# Autodesk Inventor assembly: 42146-20-03
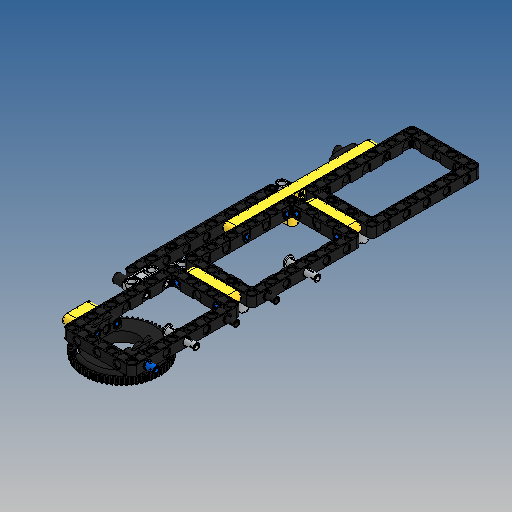
[picture p0: Inventor's stored thumbnail of the model, 512x512]
Saved by Autodesk Inventor 2025 (Build 290162010, 162A)
## iProperties
Created: 2024-11-22
Part Number: 42146-20-03
Material: Generisch
Document SubType Name: Assembly
Designer: hp.muther
Author: hp.muther
## Documents named in this file (14)
- D:\Inventor\Projekte\Muther\LEGO Technic\LEGO Technik - Raupenkran LR 13000 (42146)\42146-20-03.iam
- D:\Inventor\Projekte\Muther\LEGO Technic\LEGO Pieces\Rahmen, T-Stücke\39794-Black.ipt
- D:\Inventor\Projekte\Muther\LEGO Technic\LEGO Pieces\Pin's\2780-Black.ipt
- D:\Inventor\Projekte\Muther\LEGO Technic\LEGO Pieces\Pin's\6558-Blue.ipt
- D:\Inventor\Projekte\Muther\LEGO Technic\LEGO Pieces\Pin's\32054-LtBluishGray.ipt
- D:\Inventor\Projekte\Muther\LEGO Technic\LEGO Pieces\Lochbalken\32523-Yellow.ipt
- D:\Inventor\Projekte\Muther\LEGO Technic\LEGO Pieces\Lochbalken\32316-Yellow.ipt
- D:\Inventor\Projekte\Muther\LEGO Technic\LEGO Pieces\Lochbalken\32278-Yellow.ipt
- D:\Inventor\Projekte\Muther\LEGO Technic\LEGO Pieces\Lochbalken\771710-Black.ipt
- D:\Inventor\Projekte\Muther\LEGO Technic\LEGO Pieces\Lochbalken\40490-LtBluishGray.ipt
- D:\Inventor\Projekte\Muther\LEGO Technic\LEGO Pieces\Rund\18654-Black.ipt
- D:\Inventor\Projekte\Muther\LEGO Technic\LEGO Pieces\Verbindungselemente\48989-LtBluishGray.ipt
- D:\Inventor\Projekte\Muther\LEGO Technic\LEGO Pieces\Verbindungselemente\15461-Black.ipt
- D:\Inventor\Projekte\Muther\LEGO Technic\LEGO Pieces\Zahnrad\18938-BLACK.ipt
## Components (36 placed, 13 different names)
1. 39794-Black:1 — Einfügen:1, Einfügen:2, Einfügen:3, Einfügen:4, Passend:1, Einfügen:8, Einfügen:9, Passend:2, Passend:3, Einfügen:17, Passend:7
2. 2780-Black:1 — Einfügen:1
3. 6558-Blue:1 — Einfügen:2
4. 32054-LtBluishGray:1 — Einfügen:3
5. 18938-BLACK:1 — Einfügen:4, Passend:1
6. 32523-Yellow:1 — Einfügen:5, Einfügen:6, Einfügen:8
7. 6558-Blue:2 — Einfügen:6, Passend:3
8. 6558-Blue:3 — Einfügen:5
9. 6558-Blue:4 — Einfügen:11, Passend:4, Passend:7
10. 6558-Blue:5 — Einfügen:10
11. 39794-Black:2 — Einfügen:12, Passend:4, Einfügen:16, Passend:6, Einfügen:22, Einfügen:24, Einfügen:25, Einfügen:26, Einfügen:29, Einfügen:34
12. 32316-Yellow:1 — Einfügen:10, Einfügen:11, Einfügen:12, Einfügen:17
13. 32278-Yellow:1 — Einfügen:18, Einfügen:19, Einfügen:20, Einfügen:21, Einfügen:22, Einfügen:35, Passend:13
14. 771710-Black:1 — Einfügen:23, Passend:9, Einfügen:27, Einfügen:28, Einfügen:32
15. 40490-LtBluishGray:1 — Einfügen:34, Passend:12
16. 40490-LtBluishGray:2 — Einfügen:33, Passend:10
17. 32523-Yellow:2 — Einfügen:32, Passend:11
18. 32054-LtBluishGray:2 — Einfügen:24
19. 2780-Black:2 — Einfügen:26
20. 2780-Black:3 — Einfügen:27, Passend:12
21. 2780-Black:4 — Einfügen:28
22. 2780-Black:5 — Einfügen:25
23. 2780-Black:6 — Einfügen:29, Passend:11
24. 2780-Black:7 — Einfügen:31, Passend:10
25. 2780-Black:8 — Einfügen:30
26. 2780-Black:9 — Einfügen:18, Passend:8
27. 2780-Black:10 — Einfügen:19
28. 6558-Blue:6 — Einfügen:20, Passend:9
29. 6558-Blue:7 — Einfügen:21
30. 18654-Black:1 — Einfügen:7
31. 48989-LtBluishGray:1 — Einfügen:7, Einfügen:9, Passend:2, Einfügen:23
32. 6558-Blue:8
33. 6558-Blue:9 — Passend:6
34. 39794-Black:3 — Passend:8, Einfügen:30, Einfügen:31, Einfügen:33
35. 32316-Yellow:2 — Einfügen:16
36. 15461-Black:1 — Einfügen:35, Passend:13
## Relationships (48: Insert 35, Mate 13)
- Einfügen:1 [Insert]: 39794-Black:1 ↔ 2780-Black:1
- Einfügen:2 [Insert]: 39794-Black:1 ↔ 6558-Blue:1
- Einfügen:3 [Insert]: 39794-Black:1 ↔ 32054-LtBluishGray:1
- Einfügen:4 [Insert]: 39794-Black:1 ↔ 18938-BLACK:1
- Passend:1 [Mate]: 39794-Black:1 ↔ 18938-BLACK:1
- Einfügen:5 [Insert]: 32523-Yellow:1 ↔ 6558-Blue:3
- Einfügen:6 [Insert]: 32523-Yellow:1 ↔ 6558-Blue:2
- Einfügen:7 [Insert]: 18654-Black:1 ↔ 48989-LtBluishGray:1
- Einfügen:8 [Insert]: 39794-Black:1 ↔ 32523-Yellow:1
- Einfügen:9 [Insert]: 39794-Black:1 ↔ 48989-LtBluishGray:1
- Passend:2 [Mate]: 39794-Black:1 ↔ 48989-LtBluishGray:1
- Passend:3 [Mate]: 39794-Black:1 ↔ 6558-Blue:2
- Einfügen:10 [Insert]: 6558-Blue:5 ↔ 32316-Yellow:1
- Einfügen:11 [Insert]: 6558-Blue:4 ↔ 32316-Yellow:1
- Einfügen:12 [Insert]: 39794-Black:2 ↔ 32316-Yellow:1
- Passend:4 [Mate]: 6558-Blue:4 ↔ 39794-Black:2
- [Insert]: 6558-Blue:9 ↔ 32316-Yellow:2
- [Insert]: 6558-Blue:8 ↔ 32316-Yellow:2
- [Insert]: 39794-Black:3 ↔ 32316-Yellow:2
- [Mate]: 6558-Blue:8 ↔ 39794-Black:3
- Einfügen:16 [Insert]: 39794-Black:2 ↔ 32316-Yellow:2
- Passend:6 [Mate]: 39794-Black:2 ↔ 6558-Blue:9
- Einfügen:17 [Insert]: 39794-Black:1 ↔ 32316-Yellow:1
- Passend:7 [Mate]: 39794-Black:1 ↔ 6558-Blue:4
- Einfügen:18 [Insert]: 32278-Yellow:1 ↔ 2780-Black:9
- Einfügen:19 [Insert]: 32278-Yellow:1 ↔ 2780-Black:10
- Einfügen:20 [Insert]: 32278-Yellow:1 ↔ 6558-Blue:6
- Einfügen:21 [Insert]: 32278-Yellow:1 ↔ 6558-Blue:7
- Einfügen:22 [Insert]: 39794-Black:2 ↔ 32278-Yellow:1
- Passend:8 [Mate]: 2780-Black:9 ↔ 39794-Black:3
- Einfügen:23 [Insert]: 771710-Black:1 ↔ 48989-LtBluishGray:1
- Passend:9 [Mate]: 771710-Black:1 ↔ 6558-Blue:6
- Einfügen:24 [Insert]: 39794-Black:2 ↔ 32054-LtBluishGray:2
- Einfügen:25 [Insert]: 39794-Black:2 ↔ 2780-Black:5
- Einfügen:26 [Insert]: 39794-Black:2 ↔ 2780-Black:2
- Einfügen:27 [Insert]: 771710-Black:1 ↔ 2780-Black:3
- Einfügen:28 [Insert]: 771710-Black:1 ↔ 2780-Black:4
- Einfügen:29 [Insert]: 39794-Black:2 ↔ 2780-Black:6
- Einfügen:30 [Insert]: 2780-Black:8 ↔ 39794-Black:3
- Einfügen:31 [Insert]: 2780-Black:7 ↔ 39794-Black:3
- Einfügen:32 [Insert]: 771710-Black:1 ↔ 32523-Yellow:2
- Einfügen:33 [Insert]: 40490-LtBluishGray:2 ↔ 39794-Black:3
- Einfügen:34 [Insert]: 39794-Black:2 ↔ 40490-LtBluishGray:1
- Passend:10 [Mate]: 40490-LtBluishGray:2 ↔ 2780-Black:7
- Passend:11 [Mate]: 32523-Yellow:2 ↔ 2780-Black:6
- Passend:12 [Mate]: 40490-LtBluishGray:1 ↔ 2780-Black:3
- Einfügen:35 [Insert]: 32278-Yellow:1 ↔ 15461-Black:1
- Passend:13 [Mate]: 32278-Yellow:1 ↔ 15461-Black:1
## Named parameters: d16_d12 = 0 mm, d17_d13 = 0 mm, d18_d14 = 0 mm, d19_d15 = 0 mm
